# Autodesk Inventor assembly: v4assembly
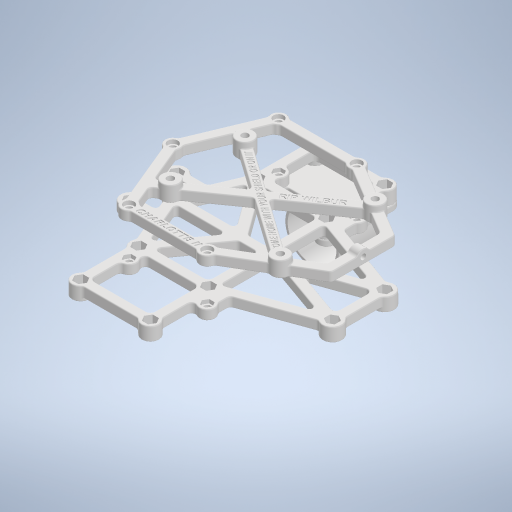
[picture p0: Inventor's stored thumbnail of the model, 512x512]
Saved by Autodesk Inventor 2024.2 (Build 282272000, 272)
## iProperties
Created: 2024-02-10
Part Number: v4assembly
Document SubType Name: Assembly
Designer: Eric
Author: Eric
## Documents named in this file (4)
- C:\Users\Eric\Desktop\scioly-robot-tour\Hardware\ipt\v4\v4assembly.iam
- C:\Users\Eric\Desktop\scioly-robot-tour\Hardware\ipt\v4\v4motormount.ipt
- C:\Users\Eric\Desktop\scioly-robot-tour\Hardware\ipt\v4\v4chassisv2.ipt
- C:\Users\Eric\Desktop\scioly-robot-tour\Hardware\ipt\v4\v4topframev3.ipt
## Components (3 placed, 3 different names)
1. v4chassisv2:1 — Mate:1, Tangent:1, Tangent:2, Flush:1
2. v4motormount:2 — Mate:1, Tangent:1, Tangent:2
3. v4topframev3:1 — Flush:2
## Relationships (5: Tangent 2, Flush 2, Mate 1)
- Mate:1: v4chassisv2:1 ↔ v4motormount:2
- Tangent:1: v4chassisv2:1 ↔ v4motormount:2
- Tangent:2: v4chassisv2:1 ↔ v4motormount:2
- Flush:1 (19 mm): v4chassisv2:1
- Flush:2: v4topframev3:1
